# Autodesk Inventor assembly: use this - gimme that tech award
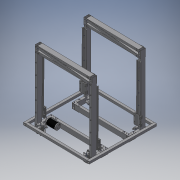
[picture p0: Inventor's stored thumbnail of the model, 180x180]
Saved by Autodesk Inventor 2018 (Build 220112000, 112)
## iProperties
Created: 2019-01-10
Part Number: use this - gimme that tech award
Document SubType Name: Assembly
Designer: maste
Author: maste
## Documents named in this file (6)
- C:\Users\maste\OneDrive\Documents\GitHub\2019CAD\Drivebase but Calvin is a mad man\use this - gimme that tech award.iam
- C:\Users\maste\OneDrive\Documents\GitHub\2019CAD\Drivebase but Calvin is a mad man\Slidey Mecanum L thing V2.iam
- C:\Users\maste\OneDrive\Documents\GitHub\2019CAD\Drivebase but Calvin is a mad man\WW_10_40_10_AL_2.ipt
- C:\Users\maste\OneDrive\Documents\GitHub\2019CAD\Drivebase but Calvin is a mad man\1x1 29in.ipt
- C:\Users\maste\OneDrive\Documents\GitHub\2019CAD\Drivebase but Calvin is a mad man\1x1 27in.ipt
- C:\Users\maste\OneDrive\Documents\GitHub\2019CAD\Drivebase but Calvin is a mad man\CIM_Motor_217-2000.ipt
## Components (11 placed, 5 different names)
1. Slidey Mecanum L thing V2:1 [sub-assembly] — Mate:59, Mate:60, Mate:61, Mate:62, Flush:1, Mate:74, Mate:75, Flush:5, Flush:6
2. Slidey Mecanum L thing V2:2 [sub-assembly] — Mate:55, Mate:56, Mate:57, Mate:58, Flush:2, Mate:72, Mate:73, Flush:3, Flush:4
3. WW_10_40_10_AL_2:1 — Mate:57, Mate:58, Flush:3
4. WW_10_40_10_AL_2:2 — Mate:59, Mate:60, Flush:5
5. WW_10_40_10_AL_2:3 — Mate:61, Mate:62, Flush:6
6. WW_10_40_10_AL_2:4 — Mate:55, Mate:56, Flush:4
7. 1x1 29in:1 — Mate:69, Mate:70, Mate:71, Mate:74, Mate:75
8. 1x1 29in:2 — Mate:63, Mate:64, Mate:65, Mate:66, Mate:67, Mate:68, Mate:72, Mate:73
9. 1x1 27in:1 — Mate:66, Mate:67, Mate:68, Mate:69, Mate:70, Mate:71, Flush:2
10. 1x1 27in:2 — Mate:63, Mate:64, Mate:65, Flush:1
11. CIM_Motor_217-2000:1
## Relationships (27: Mate 21, Flush 6)
- Mate:55: Slidey Mecanum L thing V2:2 ↔ WW_10_40_10_AL_2:4
- Mate:56: Slidey Mecanum L thing V2:2 ↔ WW_10_40_10_AL_2:4
- Mate:57: Slidey Mecanum L thing V2:2 ↔ WW_10_40_10_AL_2:1
- Mate:58: Slidey Mecanum L thing V2:2 ↔ WW_10_40_10_AL_2:1
- Mate:59: Slidey Mecanum L thing V2:1 ↔ WW_10_40_10_AL_2:2
- Mate:60: Slidey Mecanum L thing V2:1 ↔ WW_10_40_10_AL_2:2
- Mate:61: Slidey Mecanum L thing V2:1 ↔ WW_10_40_10_AL_2:3
- Mate:62: Slidey Mecanum L thing V2:1 ↔ WW_10_40_10_AL_2:3
- Mate:63: 1x1 29in:2 ↔ 1x1 27in:2
- Mate:64: 1x1 29in:2 ↔ 1x1 27in:2
- Mate:65: 1x1 29in:2 ↔ 1x1 27in:2
- Mate:66: 1x1 29in:2 ↔ 1x1 27in:1
- Mate:67: 1x1 29in:2 ↔ 1x1 27in:1
- Mate:68: 1x1 29in:2 ↔ 1x1 27in:1
- Mate:69: 1x1 29in:1 ↔ 1x1 27in:1
- Mate:70: 1x1 29in:1 ↔ 1x1 27in:1
- Mate:71: 1x1 29in:1 ↔ 1x1 27in:1
- Flush:1 (101.6 mm): Slidey Mecanum L thing V2:1 ↔ 1x1 27in:2
- Flush:2 (-101.6 mm): Slidey Mecanum L thing V2:2 ↔ 1x1 27in:1
- Mate:72 (25.4 mm): Slidey Mecanum L thing V2:2 ↔ 1x1 29in:2
- Mate:73: Slidey Mecanum L thing V2:2 ↔ 1x1 29in:2
- Mate:74: Slidey Mecanum L thing V2:1 ↔ 1x1 29in:1
- Mate:75 (25.4 mm): Slidey Mecanum L thing V2:1 ↔ 1x1 29in:1
- Flush:3: Slidey Mecanum L thing V2:2 ↔ WW_10_40_10_AL_2:1
- Flush:4: Slidey Mecanum L thing V2:2 ↔ WW_10_40_10_AL_2:4
- Flush:5: Slidey Mecanum L thing V2:1 ↔ WW_10_40_10_AL_2:2
- Flush:6: Slidey Mecanum L thing V2:1 ↔ WW_10_40_10_AL_2:3
